# Autodesk Inventor assembly: TestFitting
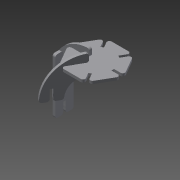
[picture p0: Inventor's stored thumbnail of the model, 180x180]
Saved by Autodesk Inventor 2015 (Build 190159000, 159)
## iProperties
Created: 2015-02-16
Part Number: TestFitting
Document SubType Name: Assembly
Designer: Iain
Author: Iain
## Documents named in this file (4)
- C:\Users\Iain\Dropbox\FabAcademy\PressFit\TestFitting.iam
- C:\Users\Iain\Dropbox\FabAcademy\PressFit\circle.ipt
- C:\Users\Iain\Dropbox\FabAcademy\PressFit\hex.ipt
- C:\Users\Iain\Dropbox\FabAcademy\PressFit\straight.ipt
## Components (4 placed, 3 different names)
1. circle:1 — Mate:1, Mate:2, Mate:3, Mate:4, Mate:12, Mate:13
2. hex:1 — Mate:1, Mate:2, Mate:9, Mate:10, Mate:11, Mate:13
3. straight:1 — Mate:3, Mate:4, Mate:12
4. circle:2 — Mate:9, Mate:10, Mate:11
## Relationships (9: Mate 9)
- Mate:1: circle:1 ↔ hex:1
- Mate:2: circle:1 ↔ hex:1
- Mate:3: circle:1 ↔ straight:1
- Mate:4: circle:1 ↔ straight:1
- Mate:9: hex:1 ↔ circle:2
- Mate:10: hex:1 ↔ circle:2
- Mate:11: hex:1 ↔ circle:2
- Mate:12: circle:1 ↔ straight:1
- Mate:13: circle:1 ↔ hex:1
